# Autodesk Inventor assembly: RT_MAIN_A_001
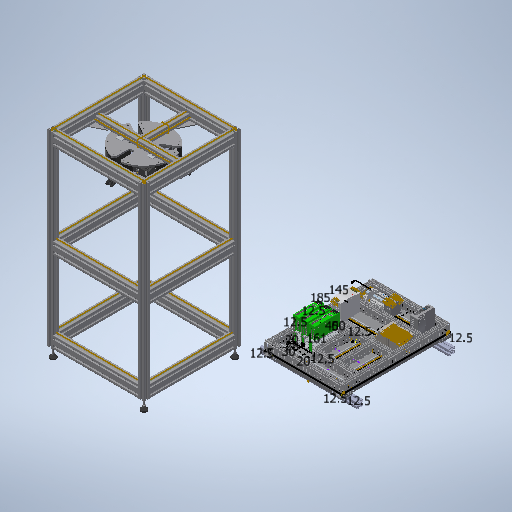
[picture p0: Inventor's stored thumbnail of the model, 512x512]
Saved by Autodesk Inventor 2025.3 (Build 293356000, 356)
## iProperties
Created: 2026-05-15
Part Number: RT_MAIN_A_001
Document SubType Name: Assembly
Designer: louis
Mass: 56308.5 g
Surface Area: 166506 cm^2
Volume: 29140.5 cm^3
Density: 1.93231 g/cm^3
Author: louis
## Documents named in this file (8)
- C:\Dev\R_Trident\02_CAD\05_Top_Assembly\RT_MAIN_A_001_V2.iam
- C:\Dev\R_Trident\02_CAD\04_Subassemblies\RT_FRM_V2_A_002_Dynamics.iam
- C:\Dev\R_Trident\02_CAD\04_Subassemblies\RT_ELE_001_ElectricalMainPlate_V0.3.iam
- C:\Dev\R_Trident\02_CAD\04_Subassemblies\RT_FRM_A_003_FrameV6.iam
- C:\Dev\R_Trident\02_CAD\05_Top_Assembly\RT_MAIN_A_001\AIP\FEA\fi7reybi8.fins
- C:\Dev\R_Trident\02_CAD\05_Top_Assembly\RT_MAIN_A_001\AIP\FEA\fi7reybi8.fsat
- C:\Dev\R_Trident\02_CAD\05_Top_Assembly\RT_MAIN_A_001\AIP\FEA\fi7reybi8.ftes
- C:\Dev\R_Trident\02_CAD\05_Top_Assembly\RT_MAIN_A_001\AIP\FEA\fi7reybi8.fwiz
## Components (3 placed, 3 different names)
1. RT_FRM_A_003_FrameV6:1 [sub-assembly] — Mate:1, Flush:1, Flush:2, Mate:2, Mate:3
2. RT_FRM_V2_A_002_Dynamics:1 [sub-assembly] — Mate:1, Mate:3, Mate:4
3. RT_ELE_001_ElectricalMainPlate_V0.3:1 [sub-assembly]
## Relationships (6: Mate 4, Flush 2)
- Mate:1: RT_FRM_A_003_FrameV6:1 ↔ RT_FRM_V2_A_002_Dynamics:1
- Flush:1: RT_FRM_A_003_FrameV6:1
- Flush:2: RT_FRM_A_003_FrameV6:1
- Mate:2: RT_FRM_A_003_FrameV6:1
- Mate:3: RT_FRM_A_003_FrameV6:1 ↔ RT_FRM_V2_A_002_Dynamics:1
- Mate:4: RT_FRM_V2_A_002_Dynamics:1
## Named parameters: sa_0 = 4500
note: some values were not read from the file. Shown as the stored number, unit unknown: "sa_0".
